# Autodesk Inventor assembly: TorsoSideUnit
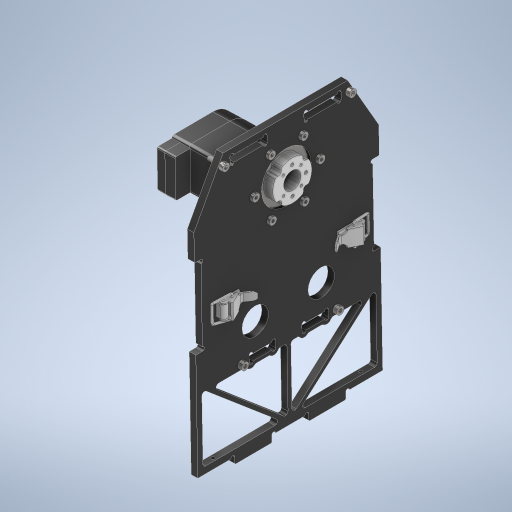
[picture p0: Inventor's stored thumbnail of the model, 512x512]
Saved by Autodesk Inventor 2024.2 (Build 282272000, 272)
## iProperties
Created: 2024-01-05
Part Number: TorsoSideUnit
Document SubType Name: Assembly
Designer: Masato Kubotera
Mass: 444.057 g
Surface Area: 821.622 cm^2
Volume: 159.843 cm^3
Density: 2.77808 g/cm^3
Author: Masato Kubotera
## Documents named in this file (9)
- C:\Users\masato\OneDrive - Chiba Institute of Technology\CIT Brains\RoboCup2024\Mechanic\SUSTAINA-OP2\NativeFiles\Boby\Torso\TorsoSideUnit.iam
- C:\Users\masato\OneDrive - Chiba Institute of Technology\CIT Brains\RoboCup2024\Mechanic\SUSTAINA-OP2\NativeFiles\Boby\COTS\Screws\CapScrew\FC-2615EB.ipt
- C:\Users\masato\OneDrive - Chiba Institute of Technology\CIT Brains\RoboCup2024\Mechanic\SUSTAINA-OP2\NativeFiles\Boby\COTS\Screws\CapScrew\UC-0310.ipt
- C:\Users\masato\OneDrive - Chiba Institute of Technology\CIT Brains\RoboCup2024\Mechanic\SUSTAINA-OP2\NativeFiles\Boby\COTS\MisumiComponents\PKWS1.iam
- C:\Users\masato\OneDrive - Chiba Institute of Technology\CIT Brains\RoboCup2024\Mechanic\SUSTAINA-OP2\NativeFiles\Boby\Torso\TorsoSideFrame_.ipt
- C:\Users\masato\OneDrive - Chiba Institute of Technology\CIT Brains\RoboCup2024\Mechanic\SUSTAINA-OP2\NativeFiles\Boby\COTS\Screws\CapScrew\UC-0308.ipt
- C:\Users\masato\OneDrive - Chiba Institute of Technology\CIT Brains\RoboCup2024\Mechanic\SUSTAINA-OP2\NativeFiles\Boby\CommonDesignedComponents\CrossRollerBearingUnit\Shoulder_CrossRollerBearingUnit.iam
- C:\Users\masato\OneDrive - Chiba Institute of Technology\CIT Brains\RoboCup2024\Mechanic\SUSTAINA-OP2\NativeFiles\Boby\COTS\Screws\LowHeadCapScrew\ULC-0306.ipt
- C:\Users\masato\OneDrive - Chiba Institute of Technology\CIT Brains\RoboCup2024\Mechanic\SUSTAINA-OP2\NativeFiles\Boby\COTS\Actuators\PMX-SCR-9204HV.ipt
## Components (17 placed, 8 different names)
1. Shoulder_CrossRollerBearingUnit:1 [sub-assembly] — Insert:17, Insert:18, Insert:3, Insert:4, Insert:256, Angle:1
2. PKWS1:1 [sub-assembly] — Insert:23, Insert:24
3. PKWS1:2 [sub-assembly] — Insert:25, Insert:26
4. TorsoSideFrame_:1 — Insert:21, Insert:22, Insert:23, Insert:24, Insert:25, Insert:26, Insert:166, Insert:167, Insert:255, Insert:256, Angle:1
5. PMX-SCR-9204HV:1 — Insert:3, Insert:4
6. UC-0308:8 — Insert:166
7. UC-0308:7 — Insert:167
8. UC-0310:2 — Insert:22
9. FC-2615EB:1 — Insert:17
10. FC-2615EB:2 — Insert:18
11. UC-0310:1 — Insert:21
12. ULC-0306:1 — Insert:255
13. ULC-0306:2
14. ULC-0306:3
15. ULC-0306:4
16. ULC-0306:5
17. ULC-0306:6
## Component patterns: (6 elements, first: ULC-0306:1)
## Relationships (15: Insert 14, Angle 1)
- Insert:3: Shoulder_CrossRollerBearingUnit:1 ↔ PMX-SCR-9204HV:1
- Insert:4: Shoulder_CrossRollerBearingUnit:1 ↔ PMX-SCR-9204HV:1
- Insert:17: Shoulder_CrossRollerBearingUnit:1 ↔ FC-2615EB:1
- Insert:18: Shoulder_CrossRollerBearingUnit:1 ↔ FC-2615EB:2
- Insert:21: TorsoSideFrame_:1 ↔ UC-0310:1
- Insert:22: TorsoSideFrame_:1 ↔ UC-0310:2
- Insert:23: PKWS1:1 ↔ TorsoSideFrame_:1
- Insert:24: PKWS1:1 ↔ TorsoSideFrame_:1
- Insert:25: PKWS1:2 ↔ TorsoSideFrame_:1
- Insert:26: PKWS1:2 ↔ TorsoSideFrame_:1
- Insert:166: TorsoSideFrame_:1 ↔ UC-0308:8
- Insert:167: TorsoSideFrame_:1 ↔ UC-0308:7
- Insert:255: TorsoSideFrame_:1 ↔ ULC-0306:1
- Insert:256: Shoulder_CrossRollerBearingUnit:1 ↔ TorsoSideFrame_:1
- Angle:1 (0 deg): Shoulder_CrossRollerBearingUnit:1 ↔ TorsoSideFrame_:1
